# Autodesk Inventor assembly: SAFRS-A-0009
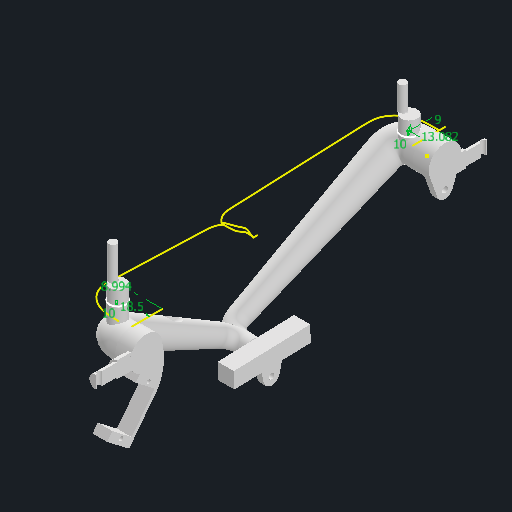
[picture p0: Inventor's stored thumbnail of the model, 512x512]
Saved by Autodesk Inventor 2026.2 (Build 302298000, 298)
## iProperties
Created: 2025-11-28
Part Number: SAFRS-A-0009
Document SubType Name: Assembly
Designer: jaewook
Author: jaewook
Title: Roll Support Left v1 Assembly
## Documents named in this file (3)
- C:\Users\jk000\OneDrive\Desktop\git\SAFRS\mechanical\inventor\02__subassemblies\roll_support_left_v1.iam
- C:\Users\jk000\OneDrive\Desktop\git\SAFRS\mechanical\inventor\01_parts\support.ipt
- C:\Users\jk000\OneDrive\Desktop\git\SAFRS\mechanical\inventor\01_parts\base_front.ipt
## Components (2 placed, 2 different names)
1. support:2 — 메이트:1
2. base_front:1 — 메이트:1
## Relationships (1: Mate 1)
- 메이트:1 [Mate]: support:2 ↔ base_front:1
